# Autodesk Inventor assembly: Assembly3
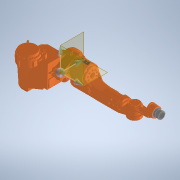
[picture p0: Inventor's stored thumbnail of the model, 180x180]
Saved by Autodesk Inventor 2021 (Build 250183000, 183)
## iProperties
Created: 2020-12-06
Part Number: Assembly3
Document SubType Name: Assembly
Designer: juanj
Mass: 39093.8 g
Surface Area: 11446.7 cm^2
Volume: 14479.2 cm^3
Density: 2.7 g/cm^3
Author: juanj
## Documents named in this file (5)
- C:\Users\juanj\OneDrive - Universidad Politécnica de Madrid\Máster\Primer semestre\Diseño y control de robots\REPOSITORIO\Robot-ABB\Assembly3.iam
- C:\Users\juanj\OneDrive - Universidad Politécnica de Madrid\Máster\Primer semestre\Diseño y control de robots\REPOSITORIO\Robot-ABB\Link3.ipt
- C:\Users\juanj\OneDrive - Universidad Politécnica de Madrid\Máster\Primer semestre\Diseño y control de robots\REPOSITORIO\Robot-ABB\link4.ipt
- C:\Users\juanj\OneDrive - Universidad Politécnica de Madrid\Máster\Primer semestre\Diseño y control de robots\REPOSITORIO\Robot-ABB\link5.ipt
- C:\Users\juanj\OneDrive - Universidad Politécnica de Madrid\Máster\Primer semestre\Diseño y control de robots\REPOSITORIO\Robot-ABB\Link6.ipt
## Components (4 placed, 4 different names)
1. Link4 — Mate:1, Mate:2, Insert:3
2. Link5 — Mate:1, Mate:2, Insert:2
3. Link6 — Insert:2
4. Link3 — Insert:3
## Relationships (4: Mate 2, Insert 2)
- Mate:1: Link4 ↔ Link5
- Mate:2: Link4 ↔ Link5
- Insert:2: Link5 ↔ Link6
- Insert:3: Link4 ↔ Link3
